# Autodesk Inventor assembly: buggy-assembly-group2
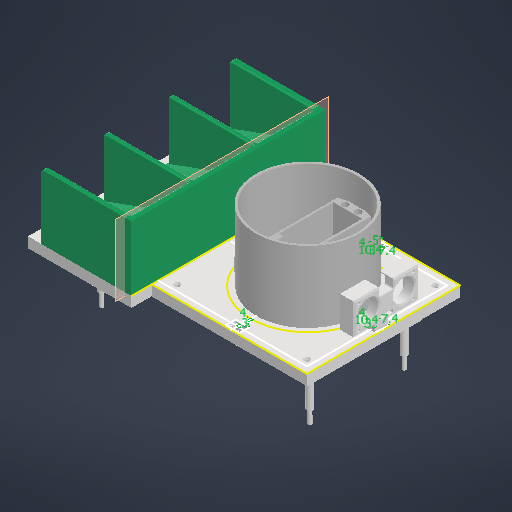
[picture p0: Inventor's stored thumbnail of the model, 512x512]
Saved by Autodesk Inventor 2026.2 (Build 302298010, 298A)
## iProperties
Created: 2026-02-23
Part Number: buggy-assembly-group2
Document SubType Name: Assembly
Designer: ts2104
Author: ts2104
## Documents named in this file (5)
- C:\Users\david\OneDrive\Documents\GitHub\System-Project-G2\mechanical\base-group2.iam
- C:\Users\david\OneDrive\Documents\GitHub\System-Project-G2\mechanical\base\rubbish-container-group2.ipt
- C:\Users\david\OneDrive\Documents\GitHub\System-Project-G2\mechanical\base\buggy-body-assembly-ready-group2.ipt
- C:\Users\david\OneDrive\Documents\GitHub\System-Project-G2\mechanical\base\us-sensor-mount-group2.ipt
- C:\Users\david\OneDrive\Documents\GitHub\System-Project-G2\mechanical\crane\rotating-base-bottom-group2.ipt
## Components (4 placed, 4 different names)
1. rubbish-container-group2:1 — Insert:1
2. buggy-body-assembly-ready-group2:1 — Mate:1, Mate:2, Mate:3, Insert:1, Mate:7, Insert:2
3. us-sensor-mount-group2:1 — Mate:7
4. rotating-base-bottom-group2:1 — Insert:2
## Relationships (6: Mate 4, Insert 2)
- Mate:1: buggy-body-assembly-ready-group2:1
- Mate:2: buggy-body-assembly-ready-group2:1
- Mate:3: buggy-body-assembly-ready-group2:1
- Insert:1: rubbish-container-group2:1 ↔ buggy-body-assembly-ready-group2:1
- Mate:7: buggy-body-assembly-ready-group2:1 ↔ us-sensor-mount-group2:1
- Insert:2: buggy-body-assembly-ready-group2:1 ↔ rotating-base-bottom-group2:1
